# Autodesk Inventor assembly: Super Gantry
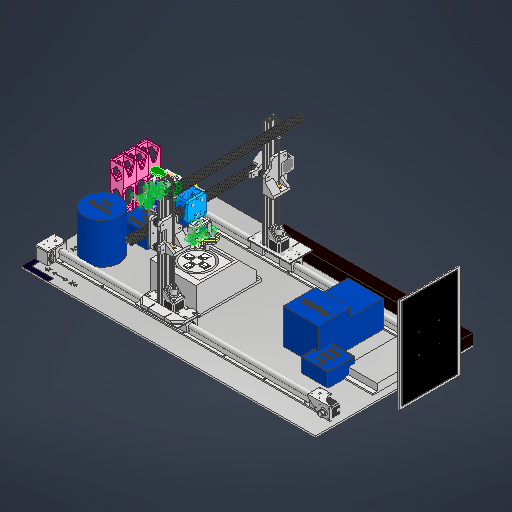
[picture p0: Inventor's stored thumbnail of the model, 512x512]
Saved by Autodesk Inventor 2025.1 (Build 291241000, 241)
## iProperties
Created: 2025-01-22
Part Number: Super Gantry
Document SubType Name: Assembly
Designer: jerem
Author: jerem
## Documents named in this file (23)
- C:\Users\jerem\Documents\GitHub\Perovskite-Automated-Synthesis-System\CAD\Gantry\Super Gantry.iam
- C:\Users\jerem\Documents\GitHub\Perovskite-Automated-Synthesis-System\CAD\Gantry\X Axis\X Axis.iam
- C:\Users\jerem\Documents\GitHub\Perovskite-Automated-Synthesis-System\CAD\Gantry\Z Axis\Z Axis.iam
- C:\Users\jerem\Documents\GitHub\Perovskite-Automated-Synthesis-System\CAD\Toolhead\Toolhead.iam
- C:\Users\jerem\Documents\GitHub\Perovskite-Automated-Synthesis-System\CAD\Camera\Camera Assembly.iam
- C:\Users\jerem\Documents\GitHub\Perovskite-Automated-Synthesis-System\CAD\Gripper\Redesign_GripperASSEM.iam
- C:\Users\jerem\Documents\GitHub\Perovskite-Automated-Synthesis-System\CAD\Non 3D Printed Parts\Spin Coater.ipt
- C:\Users\jerem\Documents\GitHub\Perovskite-Automated-Synthesis-System\CAD\Object Mounts\Spincoater Base Mount.ipt
- C:\Users\jerem\Documents\GitHub\Perovskite-Automated-Synthesis-System\CAD\Gantry\Y Axis\Y Axis.iam
- C:\Users\jerem\Documents\GitHub\Perovskite-Automated-Synthesis-System\CAD\Pipette\PipetteStand.ipt
- C:\Users\jerem\Documents\GitHub\Perovskite-Automated-Synthesis-System\CAD\Non 3D Printed Parts\Extrusion\V Extrustion 20x500mm.ipt
- C:\Users\jerem\Documents\GitHub\Perovskite-Automated-Synthesis-System\CAD\Non 3D Printed Parts\Objects\Cable Snake.ipt
- C:\Users\jerem\Documents\GitHub\Perovskite-Automated-Synthesis-System\CAD\Non 3D Printed Parts\Objects\HotPlate.ipt
- C:\Users\jerem\Documents\GitHub\Perovskite-Automated-Synthesis-System\CAD\Non 3D Printed Parts\Objects\Slide Input Tray.ipt
- C:\Users\jerem\Documents\GitHub\Perovskite-Automated-Synthesis-System\CAD\Non 3D Printed Parts\Objects\TipDropoff.ipt
- C:\Users\jerem\Documents\GitHub\Perovskite-Automated-Synthesis-System\CAD\Non 3D Printed Parts\Objects\TipPickup.ipt
- C:\Users\jerem\Documents\GitHub\Perovskite-Automated-Synthesis-System\CAD\Non 3D Printed Parts\Objects\VialCarousel.ipt
- C:\Users\jerem\Documents\GitHub\Perovskite-Automated-Synthesis-System\CAD\Non 3D Printed Parts\Objects\SpectrometerMeasurer.ipt
- C:\Users\jerem\Documents\GitHub\Perovskite-Automated-Synthesis-System\CAD\Gantry\Z Axis\Z Axis_MIR.iam
- C:\Users\jerem\Documents\GitHub\Perovskite-Automated-Synthesis-System\CAD\Pipette\NoStandAssem.iam
- C:\Users\jerem\Documents\GitHub\Perovskite-Automated-Synthesis-System\CAD\Non 3D Printed Parts\Monitor.ipt
- C:\Users\jerem\Documents\GitHub\Perovskite-Automated-Synthesis-System\CAD\Non 3D Printed Parts\Stepper Power Supply.ipt
- C:\Users\jerem\Documents\GitHub\Perovskite-Automated-Synthesis-System\CAD\Spin-Chuck\Spin-Chuck Slide.iam
## Components (24 placed, 22 different names)
1. X Axis:1 [sub-assembly] — Mate:17, Mate:25, Mate:26, Mate:27, Mate:34, Mate:41, Flush:7, Flush:8, Mate:42, Mate:43, Mate:44, Mate:45, Mate:46, Angle:2, Angle:3, Mate:47, Angle:4, Mate:48, Mate:54, Mate:55, Angle:5, Mate:59
2. Z Axis:1 [sub-assembly] — Mate:34, Mate:37, Mate:39, Flush:6, Mate:40, Angle:4
3. Toolhead:1 [sub-assembly] — Mate:8, Mate:9, Mate:10, Flush:1, Angle:1, Mate:36, Mate:51, Mate:52, Mate:53, Mate:57, Mate:58, Flush:10
4. Camera Assembly:1 [sub-assembly] — Mate:8, Mate:9, Mate:10
5. Redesign_GripperASSEM:1 [sub-assembly] — Mate:57, Mate:58, Flush:10
6. Spin Coater:1 — Mate:14, Mate:15, Mate:16, Mate:56, Flush:9
7. Spincoater Base Mount:1 — Mate:14, Mate:15, Mate:16, Mate:17, Angle:5
8. Y Axis:1 [sub-assembly] — Flush:1, Angle:1, Mate:36, Mate:37, Mate:49
9. PipetteStand:1 — Mate:26, Mate:28, Mate:29, Flush:2
10. PipetteStand:2 — Mate:25, Mate:28, Flush:2, Flush:3
11. PipetteStand:3 — Mate:27, Mate:29, Flush:3
12. V Extrustion 20x500mm:1 — Mate:39, Flush:6, Mate:40, Mate:50
13. Cable Snake:1 — Mate:41, Flush:7, Flush:8
14. HotPlate:1 — Mate:42, Mate:59
15. Slide Input Tray:1 — Mate:43
16. TipDropoff:1 — Mate:44, Angle:2
17. TipPickup:1 — Mate:45, Angle:3
18. VialCarousel:1 — Mate:46
19. SpectrometerMeasurer:1 — Mate:47
20. Z Axis_MIR:1 [sub-assembly] — Mate:48, Mate:49, Mate:50
21. NoStandAssem:1 [sub-assembly] — Mate:51, Mate:52, Mate:53
22. Monitor:1 — Mate:54
23. Stepper Power Supply:1 — Mate:55
24. Spin-Chuck Slide:1 [sub-assembly] — Mate:56, Flush:9
## Relationships (49: Mate 36, Flush 8, Angle 5)
- Mate:8: Toolhead:1 ↔ Camera Assembly:1
- Mate:9: Toolhead:1 ↔ Camera Assembly:1
- Mate:10: Toolhead:1 ↔ Camera Assembly:1
- Mate:14: Spin Coater:1 ↔ Spincoater Base Mount:1
- Mate:15: Spin Coater:1 ↔ Spincoater Base Mount:1
- Mate:16: Spin Coater:1 ↔ Spincoater Base Mount:1
- Mate:17: X Axis:1 ↔ Spincoater Base Mount:1
- Flush:1: Toolhead:1 ↔ Y Axis:1
- Mate:25: X Axis:1 ↔ PipetteStand:2
- Mate:26: X Axis:1 ↔ PipetteStand:1
- Mate:27: X Axis:1 ↔ PipetteStand:3
- Mate:28: PipetteStand:1 ↔ PipetteStand:2
- Mate:29: PipetteStand:1 ↔ PipetteStand:3
- Flush:2: PipetteStand:1 ↔ PipetteStand:2
- Flush:3: PipetteStand:2 ↔ PipetteStand:3
- Angle:1 (180 deg): Toolhead:1 ↔ Y Axis:1
- Mate:36: Toolhead:1 ↔ Y Axis:1
- Mate:34: X Axis:1 ↔ Z Axis:1
- Mate:37: Z Axis:1 ↔ Y Axis:1
- Mate:39: Z Axis:1 ↔ V Extrustion 20x500mm:1
- Flush:6: Z Axis:1 ↔ V Extrustion 20x500mm:1
- Mate:40: Z Axis:1 ↔ V Extrustion 20x500mm:1
- Mate:41: X Axis:1 ↔ Cable Snake:1
- Flush:7: X Axis:1 ↔ Cable Snake:1
- Flush:8: X Axis:1 ↔ Cable Snake:1
- Mate:42: X Axis:1 ↔ HotPlate:1
- Mate:43: X Axis:1 ↔ Slide Input Tray:1
- Mate:44: X Axis:1 ↔ TipDropoff:1
- Mate:45: X Axis:1 ↔ TipPickup:1
- Mate:46: X Axis:1 ↔ VialCarousel:1
- Angle:2 (180 deg): X Axis:1 ↔ TipDropoff:1
- Angle:3 (180 deg): X Axis:1 ↔ TipPickup:1
- Mate:47: X Axis:1 ↔ SpectrometerMeasurer:1
- Angle:4 (0 deg): X Axis:1 ↔ Z Axis:1
- Mate:48: X Axis:1 ↔ Z Axis_MIR:1
- Mate:49: Y Axis:1 ↔ Z Axis_MIR:1
- Mate:50: V Extrustion 20x500mm:1 ↔ Z Axis_MIR:1
- Mate:51: Toolhead:1 ↔ NoStandAssem:1
- Mate:52: Toolhead:1 ↔ NoStandAssem:1
- Mate:53: Toolhead:1 ↔ NoStandAssem:1
- Mate:54: X Axis:1 ↔ Monitor:1
- Mate:55: X Axis:1 ↔ Stepper Power Supply:1
- Mate:56: Spin Coater:1 ↔ Spin-Chuck Slide:1
- Flush:9: Spin Coater:1 ↔ Spin-Chuck Slide:1
- Mate:57: Toolhead:1 ↔ Redesign_GripperASSEM:1
- Mate:58: Toolhead:1 ↔ Redesign_GripperASSEM:1
- Flush:10: Toolhead:1 ↔ Redesign_GripperASSEM:1
- Angle:5 (0 deg): X Axis:1 ↔ Spincoater Base Mount:1
- Mate:59: X Axis:1 ↔ HotPlate:1
